# Autodesk Inventor assembly: Space Shelter
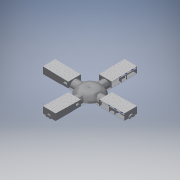
[picture p0: Inventor's stored thumbnail of the model, 180x180]
Saved by Autodesk Inventor 2017 (Build 210142000, 142)
## iProperties
Created: 2021-04-11
Part Number: Space Shelter
Document SubType Name: Assembly
Designer: udays
Author: udays
## Documents named in this file (4)
- C:\Users\udays\OneDrive\Desktop\School\Wolfhacks\Space Shelter.iam
- C:\Users\udays\OneDrive\Desktop\School\Wolfhacks\Shelter.ipt
- C:\Users\udays\OneDrive\Desktop\School\Wolfhacks\Roof.ipt
- C:\Users\udays\OneDrive\Desktop\School\Wolfhacks\Solar Panel.ipt
## Components (56 placed, 3 different names)
1. Shelter:1 — Mate:1, Flush:1, Flush:2, Mate:2, Mate:3, Mate:4, Flush:5, Angle:1
2. Shelter:2
3. Shelter:3
4. Shelter:4
5. Roof:1 — Mate:1, Flush:1, Flush:2
6. Roof:2
7. Roof:3
8. Roof:4
9. Solar Panel:1 — Mate:2, Flush:3
10. Solar Panel:2 — Mate:3, Flush:3, Flush:4
11. Solar Panel:3 — Mate:4, Flush:4
12. Solar Panel:4
13. Solar Panel:5
14. Solar Panel:6
15. Solar Panel:7
16. Solar Panel:8
17. Solar Panel:9
18. Solar Panel:10
19. Solar Panel:11
20. Solar Panel:12
21. Solar Panel:13
22. Solar Panel:14
23. Solar Panel:15
24. Solar Panel:16
25. Solar Panel:17
26. Solar Panel:18
27. Solar Panel:19
28. Solar Panel:20
29. Solar Panel:21
30. Solar Panel:22
31. Solar Panel:23
32. Solar Panel:24
33. Solar Panel:25
34. Solar Panel:26
35. Solar Panel:27
36. Solar Panel:28
37. Solar Panel:29
38. Solar Panel:30
39. Solar Panel:31
40. Solar Panel:32
41. Solar Panel:33
42. Solar Panel:34
43. Solar Panel:35
44. Solar Panel:36
45. Solar Panel:37
46. Solar Panel:38
47. Solar Panel:39
48. Solar Panel:40
49. Solar Panel:41
50. Solar Panel:42
51. Solar Panel:43
52. Solar Panel:44
53. Solar Panel:45
54. Solar Panel:46
55. Solar Panel:47
56. Solar Panel:48
## Component patterns: (4 elements, first: Shelter:1), (4 elements, first: Roof:1), (4 elements), (2 elements), Component Pattern 2:2 (2 elements), Component Pattern 2:3 (2 elements), Component Pattern 2:4 (2 elements), (2 elements, first: Solar Panel:1 + Solar Panel:2 + Solar Panel:3), Component Pattern 1:2 (2 elements), Component Pattern 1:3 (2 elements), Component Pattern 1:4 (2 elements), Component Pattern 1:5 (2 elements), Component Pattern 1:6 (2 elements), Component Pattern 1:7 (2 elements), Component Pattern 1:8 (2 elements)
## Relationships (10: Flush 5, Mate 4, Angle 1)
- Mate:1: Shelter:1 ↔ Roof:1
- Flush:1: Shelter:1 ↔ Roof:1
- Flush:2: Shelter:1 ↔ Roof:1
- Mate:2: Shelter:1 ↔ Solar Panel:1
- Mate:3: Shelter:1 ↔ Solar Panel:2
- Mate:4: Shelter:1 ↔ Solar Panel:3
- Flush:3: Solar Panel:1 ↔ Solar Panel:2
- Flush:4: Solar Panel:2 ↔ Solar Panel:3
- Flush:5 (3131.82 mm): Shelter:1
- Angle:1 (0 deg): Shelter:1
